# Autodesk Inventor assembly: ASSEMBLY_Main_Test_tube_array
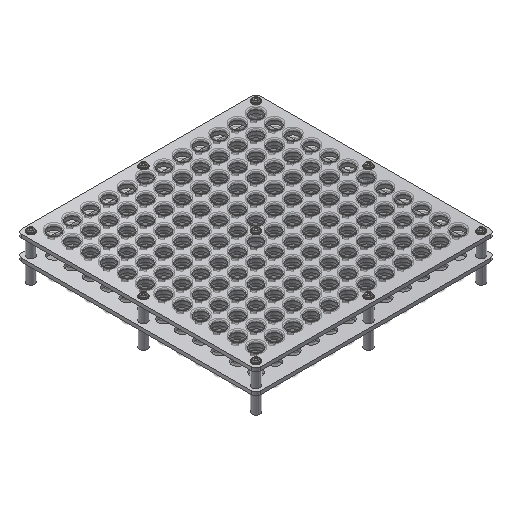
[picture p0: Inventor's stored thumbnail of the model, 512x512]
Saved by Autodesk Inventor 2025 (Build 290162010, 162A)
## iProperties
Created: 2018-06-17
Part Number: ASSEMBLY_Main_Test_tube_array
Document SubType Name: Assembly
Designer: Andrzej
Author: Andrzej
## Documents named in this file (8)
- D:\_ANDRZEJ_LACZEWSKI\_OTHER\MLTDIS - SMD parts sorting machine experimental 2 axis platform\MCAD\1_REV1\ASSEMBLY_TEST_TUBE_ARRAY_REVA\ASSEMBLY_Main_Test_tube_array.iam
- D:\_ANDRZEJ_LACZEWSKI\_OTHER\MLTDIS - SMD parts sorting machine experimental 2 axis platform\MCAD\1_REV1\ASSEMBLY_TEST_TUBE_ARRAY_REVA\3DP_PLA_Test_tube_array_bottom_plate.ipt
- D:\_ANDRZEJ_LACZEWSKI\_OTHER\MLTDIS - SMD parts sorting machine experimental 2 axis platform\MCAD\1_REV1\ASSEMBLY_TEST_TUBE_ARRAY_REVA\3DP_PLA_Test_tube_array_top_plate.ipt
- D:\_ANDRZEJ_LACZEWSKI\_OTHER\MLTDIS - SMD parts sorting machine experimental 2 axis platform\MCAD\1_REV1\__COTS_PARTS\COTS_Eppendorf_10ml_test_tube.ipt
- D:\_ANDRZEJ_LACZEWSKI\_OTHER\MLTDIS - SMD parts sorting machine experimental 2 axis platform\MCAD\1_REV1\ASSEMBLY_TEST_TUBE_ARRAY_REVA\3DP_PLA_Test_tube_array_top_spacer.ipt
- D:\_ANDRZEJ_LACZEWSKI\_OTHER\MLTDIS - SMD parts sorting machine experimental 2 axis platform\MCAD\1_REV1\ASSEMBLY_TEST_TUBE_ARRAY_REVA\3DP_PLA_Test_tube_array_bottom_spacer.ipt
- D:\_ANDRZEJ_LACZEWSKI\_OTHER\MLTDIS - SMD parts sorting machine experimental 2 axis platform\MCAD\1_REV1\__CONTENT_CENTER_PARTS\en-US\DIN 125-2  A\DIN 125-2 - A 3,2A.ipt
- D:\_ANDRZEJ_LACZEWSKI\_OTHER\MLTDIS - SMD parts sorting machine experimental 2 axis platform\MCAD\1_REV1\__CONTENT_CENTER_PARTS\en-US\AS 1427(05)\AS 1427 - M3 x 40(5) II.ipt
## Components (182 placed, 7 different names)
1. 3DP_PLA_Test_tube_array_bottom_plate:1 — Flush:1, Flush:2, Mate:1, Mate:4, Mate:5, Mate:6, Mate:7
2. 3DP_PLA_Test_tube_array_top_plate:1 — Flush:1, Flush:2, Mate:1, Mate:2, Mate:3, Mate:8, Mate:9, Mate:10, Mate:11, Mate:12, Mate:13, Mate:14, Mate:15, Mate:16, Mate:17, Mate:18, Mate:19, Mate:20, Mate:21, Mate:22, Mate:23, Mate:24, Mate:25
3. AS 1427 H - Metric M3 x 40:9 — Insert:9
4. AS 1427 H - Metric M3 x 40:8 — Insert:8
5. AS 1427 H - Metric M3 x 40:7 — Insert:7
6. AS 1427 H - Metric M3 x 40:6 — Insert:6
7. AS 1427 H - Metric M3 x 40:5 — Insert:5
8. AS 1427 H - Metric M3 x 40:4 — Insert:4
9. AS 1427 H - Metric M3 x 40:3 — Insert:3
10. AS 1427 H - Metric M3 x 40:2 — Insert:2
11. DIN 125-2 A A 3,2:9 — Mate:24, Mate:25, Insert:9
12. DIN 125-2 A A 3,2:8 — Mate:22, Mate:23, Insert:8
13. DIN 125-2 A A 3,2:7 — Mate:20, Mate:21, Insert:7
14. DIN 125-2 A A 3,2:6 — Mate:18, Mate:19, Insert:6
15. DIN 125-2 A A 3,2:5 — Mate:16, Mate:17, Insert:5
16. DIN 125-2 A A 3,2:4 — Mate:14, Mate:15, Insert:4
17. DIN 125-2 A A 3,2:3 — Mate:12, Mate:13, Insert:3
18. DIN 125-2 A A 3,2:2 — Mate:10, Mate:11, Insert:2
19. AS 1427 H - Metric M3 x 40:1 — Insert:1
20. DIN 125-2 A A 3,2:1 — Mate:8, Mate:9, Insert:1
21. COTS_Eppendorf_10ml_test_tube:1 — Mate:2, Mate:3
22. COTS_Eppendorf_10ml_test_tube:2
23. COTS_Eppendorf_10ml_test_tube:3
24. COTS_Eppendorf_10ml_test_tube:4
25. COTS_Eppendorf_10ml_test_tube:5
26. COTS_Eppendorf_10ml_test_tube:6
27. COTS_Eppendorf_10ml_test_tube:7
28. COTS_Eppendorf_10ml_test_tube:8
29. COTS_Eppendorf_10ml_test_tube:9
30. COTS_Eppendorf_10ml_test_tube:10
31. COTS_Eppendorf_10ml_test_tube:11
32. COTS_Eppendorf_10ml_test_tube:12
33. COTS_Eppendorf_10ml_test_tube:13
34. COTS_Eppendorf_10ml_test_tube:14
35. COTS_Eppendorf_10ml_test_tube:15
36. COTS_Eppendorf_10ml_test_tube:16
37. COTS_Eppendorf_10ml_test_tube:17
38. COTS_Eppendorf_10ml_test_tube:18
39. COTS_Eppendorf_10ml_test_tube:19
40. COTS_Eppendorf_10ml_test_tube:20
41. COTS_Eppendorf_10ml_test_tube:21
42. COTS_Eppendorf_10ml_test_tube:22
43. COTS_Eppendorf_10ml_test_tube:23
44. COTS_Eppendorf_10ml_test_tube:24
45. COTS_Eppendorf_10ml_test_tube:25
46. COTS_Eppendorf_10ml_test_tube:26
47. COTS_Eppendorf_10ml_test_tube:27
48. COTS_Eppendorf_10ml_test_tube:28
49. COTS_Eppendorf_10ml_test_tube:29
50. COTS_Eppendorf_10ml_test_tube:30
51. COTS_Eppendorf_10ml_test_tube:31
52. COTS_Eppendorf_10ml_test_tube:32
53. COTS_Eppendorf_10ml_test_tube:33
54. COTS_Eppendorf_10ml_test_tube:34
55. COTS_Eppendorf_10ml_test_tube:35
56. COTS_Eppendorf_10ml_test_tube:36
57. COTS_Eppendorf_10ml_test_tube:37
58. COTS_Eppendorf_10ml_test_tube:38
59. COTS_Eppendorf_10ml_test_tube:39
60. COTS_Eppendorf_10ml_test_tube:40
61. COTS_Eppendorf_10ml_test_tube:41
62. COTS_Eppendorf_10ml_test_tube:42
63. COTS_Eppendorf_10ml_test_tube:43
64. COTS_Eppendorf_10ml_test_tube:44
65. COTS_Eppendorf_10ml_test_tube:45
66. COTS_Eppendorf_10ml_test_tube:46
67. COTS_Eppendorf_10ml_test_tube:47
68. COTS_Eppendorf_10ml_test_tube:48
69. COTS_Eppendorf_10ml_test_tube:49
70. COTS_Eppendorf_10ml_test_tube:50
71. COTS_Eppendorf_10ml_test_tube:51
72. COTS_Eppendorf_10ml_test_tube:52
73. COTS_Eppendorf_10ml_test_tube:53
74. COTS_Eppendorf_10ml_test_tube:54
75. COTS_Eppendorf_10ml_test_tube:55
76. COTS_Eppendorf_10ml_test_tube:56
77. COTS_Eppendorf_10ml_test_tube:57
78. COTS_Eppendorf_10ml_test_tube:58
79. COTS_Eppendorf_10ml_test_tube:59
80. COTS_Eppendorf_10ml_test_tube:60
81. COTS_Eppendorf_10ml_test_tube:61
82. COTS_Eppendorf_10ml_test_tube:62
83. COTS_Eppendorf_10ml_test_tube:63
84. COTS_Eppendorf_10ml_test_tube:64
85. COTS_Eppendorf_10ml_test_tube:65
86. COTS_Eppendorf_10ml_test_tube:66
87. COTS_Eppendorf_10ml_test_tube:67
88. COTS_Eppendorf_10ml_test_tube:68
89. COTS_Eppendorf_10ml_test_tube:69
90. COTS_Eppendorf_10ml_test_tube:70
91. COTS_Eppendorf_10ml_test_tube:71
92. COTS_Eppendorf_10ml_test_tube:72
93. COTS_Eppendorf_10ml_test_tube:73
94. COTS_Eppendorf_10ml_test_tube:74
95. COTS_Eppendorf_10ml_test_tube:75
96. COTS_Eppendorf_10ml_test_tube:76
97. COTS_Eppendorf_10ml_test_tube:77
98. COTS_Eppendorf_10ml_test_tube:78
99. COTS_Eppendorf_10ml_test_tube:79
100. COTS_Eppendorf_10ml_test_tube:80
101. COTS_Eppendorf_10ml_test_tube:81
102. COTS_Eppendorf_10ml_test_tube:82
103. COTS_Eppendorf_10ml_test_tube:83
104. COTS_Eppendorf_10ml_test_tube:84
105. COTS_Eppendorf_10ml_test_tube:85
106. COTS_Eppendorf_10ml_test_tube:86
107. COTS_Eppendorf_10ml_test_tube:87
108. COTS_Eppendorf_10ml_test_tube:88
109. COTS_Eppendorf_10ml_test_tube:89
110. COTS_Eppendorf_10ml_test_tube:90
111. COTS_Eppendorf_10ml_test_tube:91
112. COTS_Eppendorf_10ml_test_tube:92
113. COTS_Eppendorf_10ml_test_tube:93
114. COTS_Eppendorf_10ml_test_tube:94
115. COTS_Eppendorf_10ml_test_tube:95
116. COTS_Eppendorf_10ml_test_tube:96
117. COTS_Eppendorf_10ml_test_tube:97
118. COTS_Eppendorf_10ml_test_tube:98
119. COTS_Eppendorf_10ml_test_tube:99
120. COTS_Eppendorf_10ml_test_tube:100
121. COTS_Eppendorf_10ml_test_tube:101
122. COTS_Eppendorf_10ml_test_tube:102
123. COTS_Eppendorf_10ml_test_tube:103
124. COTS_Eppendorf_10ml_test_tube:104
125. COTS_Eppendorf_10ml_test_tube:105
126. COTS_Eppendorf_10ml_test_tube:106
127. COTS_Eppendorf_10ml_test_tube:107
128. COTS_Eppendorf_10ml_test_tube:108
129. COTS_Eppendorf_10ml_test_tube:109
130. COTS_Eppendorf_10ml_test_tube:110
131. COTS_Eppendorf_10ml_test_tube:111
132. COTS_Eppendorf_10ml_test_tube:112
133. COTS_Eppendorf_10ml_test_tube:113
134. COTS_Eppendorf_10ml_test_tube:114
135. COTS_Eppendorf_10ml_test_tube:115
136. COTS_Eppendorf_10ml_test_tube:116
137. COTS_Eppendorf_10ml_test_tube:117
138. COTS_Eppendorf_10ml_test_tube:118
139. COTS_Eppendorf_10ml_test_tube:119
140. COTS_Eppendorf_10ml_test_tube:120
141. COTS_Eppendorf_10ml_test_tube:121
142. COTS_Eppendorf_10ml_test_tube:122
143. COTS_Eppendorf_10ml_test_tube:123
144. COTS_Eppendorf_10ml_test_tube:124
145. COTS_Eppendorf_10ml_test_tube:125
146. COTS_Eppendorf_10ml_test_tube:126
147. COTS_Eppendorf_10ml_test_tube:127
148. COTS_Eppendorf_10ml_test_tube:128
149. COTS_Eppendorf_10ml_test_tube:129
150. COTS_Eppendorf_10ml_test_tube:130
151. COTS_Eppendorf_10ml_test_tube:131
152. COTS_Eppendorf_10ml_test_tube:132
153. COTS_Eppendorf_10ml_test_tube:133
154. COTS_Eppendorf_10ml_test_tube:134
155. COTS_Eppendorf_10ml_test_tube:135
156. COTS_Eppendorf_10ml_test_tube:136
157. COTS_Eppendorf_10ml_test_tube:137
158. COTS_Eppendorf_10ml_test_tube:138
159. COTS_Eppendorf_10ml_test_tube:139
160. COTS_Eppendorf_10ml_test_tube:140
161. COTS_Eppendorf_10ml_test_tube:141
162. COTS_Eppendorf_10ml_test_tube:142
163. COTS_Eppendorf_10ml_test_tube:143
164. COTS_Eppendorf_10ml_test_tube:144
165. 3DP_PLA_Test_tube_array_top_spacer:6 — Mate:4, Mate:5
166. 3DP_PLA_Test_tube_array_top_spacer:7
167. 3DP_PLA_Test_tube_array_top_spacer:8
168. 3DP_PLA_Test_tube_array_top_spacer:9
169. 3DP_PLA_Test_tube_array_top_spacer:10
170. 3DP_PLA_Test_tube_array_top_spacer:11
171. 3DP_PLA_Test_tube_array_top_spacer:12
172. 3DP_PLA_Test_tube_array_top_spacer:13
173. 3DP_PLA_Test_tube_array_top_spacer:14
174. 3DP_PLA_Test_tube_array_bottom_spacer:1 — Mate:6, Mate:7
175. 3DP_PLA_Test_tube_array_bottom_spacer:2
176. 3DP_PLA_Test_tube_array_bottom_spacer:3
177. 3DP_PLA_Test_tube_array_bottom_spacer:4
178. 3DP_PLA_Test_tube_array_bottom_spacer:5
179. 3DP_PLA_Test_tube_array_bottom_spacer:6
180. 3DP_PLA_Test_tube_array_bottom_spacer:7
181. 3DP_PLA_Test_tube_array_bottom_spacer:8
182. 3DP_PLA_Test_tube_array_bottom_spacer:9
## Component patterns: (144 elements, first: COTS_Eppendorf_10ml_test_tube:1), (9 elements, first: 3DP_PLA_Test_tube_array_top_spacer:6), (9 elements, first: 3DP_PLA_Test_tube_array_bottom_spacer:1)
## Relationships (36: Mate 25, Insert 9, Flush 2)
- Flush:1: 3DP_PLA_Test_tube_array_bottom_plate:1 ↔ 3DP_PLA_Test_tube_array_top_plate:1
- Flush:2: 3DP_PLA_Test_tube_array_bottom_plate:1 ↔ 3DP_PLA_Test_tube_array_top_plate:1
- Mate:1 (15 mm): 3DP_PLA_Test_tube_array_bottom_plate:1 ↔ 3DP_PLA_Test_tube_array_top_plate:1
- Mate:2: 3DP_PLA_Test_tube_array_top_plate:1 ↔ COTS_Eppendorf_10ml_test_tube:1
- Mate:3: 3DP_PLA_Test_tube_array_top_plate:1 ↔ COTS_Eppendorf_10ml_test_tube:1
- Mate:4: 3DP_PLA_Test_tube_array_bottom_plate:1 ↔ 3DP_PLA_Test_tube_array_top_spacer:6
- Mate:5: 3DP_PLA_Test_tube_array_bottom_plate:1 ↔ 3DP_PLA_Test_tube_array_top_spacer:6
- Mate:6: 3DP_PLA_Test_tube_array_bottom_plate:1 ↔ 3DP_PLA_Test_tube_array_bottom_spacer:1
- Mate:7: 3DP_PLA_Test_tube_array_bottom_plate:1 ↔ 3DP_PLA_Test_tube_array_bottom_spacer:1
- Mate:8: 3DP_PLA_Test_tube_array_top_plate:1 ↔ DIN 125-2 A A 3,2:1
- Mate:9: 3DP_PLA_Test_tube_array_top_plate:1 ↔ DIN 125-2 A A 3,2:1
- Mate:10: 3DP_PLA_Test_tube_array_top_plate:1 ↔ DIN 125-2 A A 3,2:2
- Mate:11: 3DP_PLA_Test_tube_array_top_plate:1 ↔ DIN 125-2 A A 3,2:2
- Mate:12: 3DP_PLA_Test_tube_array_top_plate:1 ↔ DIN 125-2 A A 3,2:3
- Mate:13: 3DP_PLA_Test_tube_array_top_plate:1 ↔ DIN 125-2 A A 3,2:3
- Mate:14: 3DP_PLA_Test_tube_array_top_plate:1 ↔ DIN 125-2 A A 3,2:4
- Mate:15: 3DP_PLA_Test_tube_array_top_plate:1 ↔ DIN 125-2 A A 3,2:4
- Mate:16: 3DP_PLA_Test_tube_array_top_plate:1 ↔ DIN 125-2 A A 3,2:5
- Mate:17: 3DP_PLA_Test_tube_array_top_plate:1 ↔ DIN 125-2 A A 3,2:5
- Mate:18: 3DP_PLA_Test_tube_array_top_plate:1 ↔ DIN 125-2 A A 3,2:6
- Mate:19: 3DP_PLA_Test_tube_array_top_plate:1 ↔ DIN 125-2 A A 3,2:6
- Mate:20: 3DP_PLA_Test_tube_array_top_plate:1 ↔ DIN 125-2 A A 3,2:7
- Mate:21: 3DP_PLA_Test_tube_array_top_plate:1 ↔ DIN 125-2 A A 3,2:7
- Mate:22: 3DP_PLA_Test_tube_array_top_plate:1 ↔ DIN 125-2 A A 3,2:8
- Mate:23: 3DP_PLA_Test_tube_array_top_plate:1 ↔ DIN 125-2 A A 3,2:8
- Mate:24: 3DP_PLA_Test_tube_array_top_plate:1 ↔ DIN 125-2 A A 3,2:9
- Mate:25: 3DP_PLA_Test_tube_array_top_plate:1 ↔ DIN 125-2 A A 3,2:9
- Insert:1: AS 1427 H - Metric M3 x 40:1 ↔ DIN 125-2 A A 3,2:1
- Insert:2: AS 1427 H - Metric M3 x 40:2 ↔ DIN 125-2 A A 3,2:2
- Insert:3: AS 1427 H - Metric M3 x 40:3 ↔ DIN 125-2 A A 3,2:3
- Insert:4: AS 1427 H - Metric M3 x 40:4 ↔ DIN 125-2 A A 3,2:4
- Insert:5: AS 1427 H - Metric M3 x 40:5 ↔ DIN 125-2 A A 3,2:5
- Insert:6: AS 1427 H - Metric M3 x 40:6 ↔ DIN 125-2 A A 3,2:6
- Insert:7: AS 1427 H - Metric M3 x 40:7 ↔ DIN 125-2 A A 3,2:7
- Insert:8: AS 1427 H - Metric M3 x 40:8 ↔ DIN 125-2 A A 3,2:8
- Insert:9: AS 1427 H - Metric M3 x 40:9 ↔ DIN 125-2 A A 3,2:9
